# Autodesk Inventor assembly: WheelAssembly3.0
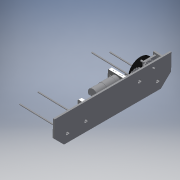
[picture p0: Inventor's stored thumbnail of the model, 180x180]
Saved by Autodesk Inventor 2017 (Build 210142000, 142)
## iProperties
Created: 2017-07-22
Part Number: WheelAssembly3.0
Document SubType Name: Assembly
Designer: User
Author: User
## Documents named in this file (13)
- C:\Robotics\CAD\WheelAssembly3.0.iam
- C:\Robotics\CAD\2016-17_CAD\DriveTrain\DriveTrain3.0.ipt
- C:\Robotics\CAD\COTSParts\Motors\Andymark 2964  NeveRest 40 Motor.ipt
- C:\Robotics\CAD\COTSParts\Tetrix\tetrix-motor-mounts-1.snapshot.1\Tetrex 2pc motor mount.ipt
- C:\Robotics\CAD\COTSParts\Actobotics\615 parts\615398.ipt
- C:\Robotics\CAD\2016-17_CAD\Custom COTS\4inax.ipt
- C:\Robotics\CAD\COTSParts\Actobotics\615 parts\615106.ipt
- C:\Robotics\CAD\COTSParts\Actobotics\545 parts\545556.ipt
- C:\Robotics\CAD\COTSParts\Actobotics\615 parts\615114.ipt
- C:\Robotics\CAD\2016-17_CAD\Mechanum Wheel Adapter.ipt
- C:\Robotics\CAD\2016-17_CAD\DriveTrain\Tensioner.iam
- C:\Robotics\CAD\COTSParts\Actobotics\545 parts\545456.ipt
- C:\Robotics\CAD\COTSParts\Wheels\4in Wheel Intergreated Hub 8mm Rev2.ipt
## Components (26 placed, 12 different names)
1. DriveTrain3.0:1 — Flush:3, Flush:4, Mate:2, Flush:5, Mate:3, Flush:6, Angle:1, Insert:7, Insert:8, Angle:2, Insert:9, Insert:10, Insert:16, Insert:17, Mate:6, Flush:9, Flush:10
2. Andymark 2964  NeveRest 40 Motor:1 — Insert:3, Insert:6, Angle:2
3. Andymark 2964  NeveRest 40 Motor:2 — Insert:4, Insert:5, Angle:1
4. Tetrex 2pc motor mount:1 — Insert:3, Flush:3, Mate:3, Flush:6
5. Tetrex 2pc motor mount:2 — Insert:4, Flush:4, Mate:2, Flush:5
6. 615398:1 — Insert:5
7. 615398:2 — Insert:6
8. 615398:3 — Insert:7
9. 615398:4 — Insert:8
10. 4inax:1 — Insert:9, Mate:4
11. 4inax:2 — Insert:10, Mate:7
12. 615106:1 — Insert:13, Flush:7, Mate:7, Flush:11
13. 615106:2 — Insert:20, Flush:8
14. 545556:1 — Insert:13, Insert:22
15. 545556:2 — Insert:14
16. 615114:1 — Mate:4, Flush:7, Insert:14
17. Mechanum Wheel Adapter:1
18. 4inax:3 — Insert:16, Mate:5
19. 4inax:4 — Insert:17
20. 545556:3 — Insert:20
21. 615114:2 — Mate:5, Flush:8, Insert:21
22. 545556:4 — Insert:21
23. Tensioner:1 [sub-assembly] — Mate:6, Flush:9, Flush:10, Flush:11
24. 545556:5 — Insert:22, Insert:23
25. 545456:1 — Insert:23, Insert:24
26. 4in Wheel Intergreated Hub 8mm Rev2:1 — Insert:24
## Relationships (34: Insert 17, Flush 9, Mate 6, Angle 2)
- Insert:3: Andymark 2964  NeveRest 40 Motor:1 ↔ Tetrex 2pc motor mount:1
- Insert:4: Andymark 2964  NeveRest 40 Motor:2 ↔ Tetrex 2pc motor mount:2
- Flush:3 (159.5374 mm): DriveTrain3.0:1 ↔ Tetrex 2pc motor mount:1
- Flush:4 (159.5374 mm): DriveTrain3.0:1 ↔ Tetrex 2pc motor mount:2
- Insert:5: Andymark 2964  NeveRest 40 Motor:2 ↔ 615398:1
- Mate:2: DriveTrain3.0:1 ↔ Tetrex 2pc motor mount:2
- Flush:5 (7.3152 mm): DriveTrain3.0:1 ↔ Tetrex 2pc motor mount:2
- Mate:3: DriveTrain3.0:1 ↔ Tetrex 2pc motor mount:1
- Flush:6 (-20.3454 mm): DriveTrain3.0:1 ↔ Tetrex 2pc motor mount:1
- Angle:1 (0 deg): DriveTrain3.0:1 ↔ Andymark 2964  NeveRest 40 Motor:2
- Insert:6: Andymark 2964  NeveRest 40 Motor:1 ↔ 615398:2
- Insert:7 (25.4508 mm): DriveTrain3.0:1 ↔ 615398:3
- Insert:8 (25.4508 mm): DriveTrain3.0:1 ↔ 615398:4
- Angle:2 (180 deg): DriveTrain3.0:1 ↔ Andymark 2964  NeveRest 40 Motor:1
- Insert:9 (-6.35 mm): DriveTrain3.0:1 ↔ 4inax:1
- Insert:10 (-6.35 mm): DriveTrain3.0:1 ↔ 4inax:2
- Insert:13: 615106:1 ↔ 545556:1
- Mate:4: 4inax:1 ↔ 615114:1
- Flush:7: 615106:1 ↔ 615114:1
- Insert:14: 545556:2 ↔ 615114:1
- Insert:16 (-6.35 mm): DriveTrain3.0:1 ↔ 4inax:3
- Insert:17 (-6.35 mm): DriveTrain3.0:1 ↔ 4inax:4
- Insert:20: 615106:2 ↔ 545556:3
- Mate:5: 4inax:3 ↔ 615114:2
- Flush:8: 615106:2 ↔ 615114:2
- Insert:21: 615114:2 ↔ 545556:4
- Mate:6: DriveTrain3.0:1 ↔ Tensioner:1
- Flush:9 (26.035 mm): DriveTrain3.0:1 ↔ Tensioner:1
- Flush:10 (-1.905 mm): DriveTrain3.0:1 ↔ Tensioner:1
- Mate:7: 4inax:2 ↔ 615106:1
- Flush:11: 615106:1 ↔ Tensioner:1
- Insert:22 (9.525 mm): 545556:1 ↔ 545556:5
- Insert:23: 545556:5 ↔ 545456:1
- Insert:24: 545456:1 ↔ 4in Wheel Intergreated Hub 8mm Rev2:1
